# Autodesk Inventor assembly: Slider_crank_mechanism
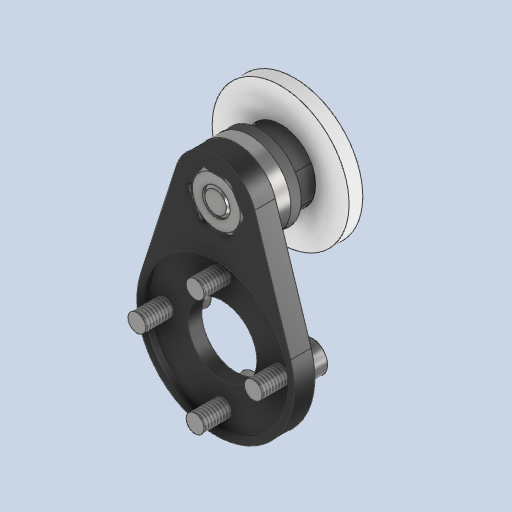
[picture p0: Inventor's stored thumbnail of the model, 512x512]
Saved by Autodesk Inventor 2022.3 (Build 263350000, 350)
## iProperties
Created: 2022-06-15
Part Number: Slider_crank_mechanism
Document SubType Name: Assembly
Designer: Masato Kubotera
Author: Masato Kubotera
## Documents named in this file (9)
- C:\Users\Masato\Desktop\SUSTAINA-OP\LowerBody\Slider_crank\Slider_crank_mechanism.iam
- C:\Users\Masato\Desktop\SUSTAINA-OP\LowerBody\Slider_crank\Slider_crank_horn.ipt
- C:\Users\Masato\Desktop\SUSTAINA-OP\ReadyMade\InsertNut\S4-05-3W.ipt
- C:\Users\Masato\Desktop\SUSTAINA-OP\ReadyMade\Washer\TT-1020-20.ipt
- C:\Users\Masato\Desktop\SUSTAINA-OP\ReadyMade\Washer\UUW-0614-05BH.ipt
- C:\Users\Masato\Desktop\SUSTAINA-OP\ReadyMade\Bush\LED-0606.ipt
- C:\Users\Masato\Desktop\SUSTAINA-OP\ReadyMade\Washer\UUW-0412-20H.ipt
- C:\Users\Masato\Desktop\SUSTAINA-OP\ReadyMade\Screw\DBTS4-7-5-DHC.ipt
- C:\Users\Masato\Desktop\SUSTAINA-OP\ReadyMade\Screw\UC-2606.ipt
## Components (11 placed, 8 different names)
1. UUW-0412-20H:1 — Insert:11, Insert:12, Insert:14
2. DBTS4-7-5-DHC:1 — Insert:13, Insert:14
3. Slider_crank_horn:1 — フラッシュ:1, フラッシュ:2, フラッシュ:3, 挿入:1, 角度:1, 角度:2, Insert:11, Insert:15, Insert:16, Insert:17, Insert:18
4. S4-05-3W:1 — 挿入:1, 角度:1
5. TT-1020-20:1 — 挿入:6
6. UUW-0614-05BH:1 — 挿入:6, Insert:13
7. LED-0606:1 — 角度:2, Insert:12
8. UC-2606:1 — Insert:15
9. UC-2606:2 — Insert:16
10. UC-2606:3 — Insert:17
11. UC-2606:4 — Insert:18
## Relationships (15: Insert 10, Flush 3, Angle 2)
- フラッシュ:1 [Flush]: Slider_crank_horn:1
- フラッシュ:2 [Flush]: Slider_crank_horn:1
- フラッシュ:3 [Flush]: Slider_crank_horn:1
- 挿入:1 [Insert]: Slider_crank_horn:1 ↔ S4-05-3W:1
- 角度:1 [Angle] (0 deg): Slider_crank_horn:1 ↔ S4-05-3W:1
- 角度:2 [Angle] (0 deg): Slider_crank_horn:1 ↔ LED-0606:1
- 挿入:6 [Insert]: TT-1020-20:1 ↔ UUW-0614-05BH:1
- Insert:11: UUW-0412-20H:1 ↔ Slider_crank_horn:1
- Insert:12: UUW-0412-20H:1 ↔ LED-0606:1
- Insert:13: DBTS4-7-5-DHC:1 ↔ UUW-0614-05BH:1
- Insert:14: UUW-0412-20H:1 ↔ DBTS4-7-5-DHC:1
- Insert:15: Slider_crank_horn:1 ↔ UC-2606:1
- Insert:16: Slider_crank_horn:1 ↔ UC-2606:2
- Insert:17: Slider_crank_horn:1 ↔ UC-2606:3
- Insert:18: Slider_crank_horn:1 ↔ UC-2606:4
